# Autodesk Inventor assembly: BODY
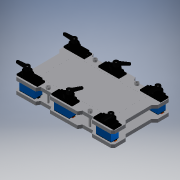
[picture p0: Inventor's stored thumbnail of the model, 180x180]
Saved by Autodesk Inventor 2017 (Build 210142000, 142)
## iProperties
Created: 2017-09-24
Part Number: BODY
Document SubType Name: Assembly
Designer: Alexander Miller
Author: Alexander Miller
## Documents named in this file (8)
- X:\Alex\Documents\Git\HeRo-Mini\Hardware\BODY.iam
- X:\Alex\Documents\Git\HeRo-Mini\Hardware\BODY_BOTTOM.ipt
- X:\Alex\Documents\Git\HeRo-Mini\Hardware\BODY_TOP.ipt
- X:\Alex\Documents\Git\HeRo-Mini\Hardware\SERVO.iam
- X:\Alex\Documents\Git\HeRo-Mini\Hardware\BODY_TOP_COVER.ipt
- X:\Alex\Documents\Git\HeRo-Mini\Hardware\MAGNET.ipt
- X:\Alex\Documents\Git\HeRo-Mini\Hardware\NUT_3MM.ipt
- X:\Alex\Documents\Git\HeRo-Mini\Hardware\M3_SCREW_25MM.ipt
## Components (35 placed, 7 different names)
1. BODY_BOTTOM:1 — Rigid:8, Rigid:9, Rigid:10, Rigid:11, Rigid:12, Rigid:13, Rigid:22, Rigid:23, Rigid:24, Rigid:25, Rigid:26, Rigid:27, Rigid:28, Rigid:29, Rigid:34, Rigid:35, Rigid:36, Rigid:37, Rigid:38, Rigid:39
2. BODY_TOP:1 — Rigid:7, Rigid:14, Rigid:15, Rigid:16, Rigid:17, Rigid:30, Rigid:31, Rigid:32, Rigid:33
3. SERVO:1 [sub-assembly] — Rigid:7, Rigid:13
4. SERVO:2 [sub-assembly] — Rigid:12
5. SERVO:3 [sub-assembly] — Rigid:11
6. SERVO:4 [sub-assembly] — Rigid:10
7. SERVO:5 [sub-assembly] — Rigid:9
8. SERVO:6 [sub-assembly] — Rigid:8
9. BODY_TOP_COVER:1 — Rigid:18, Rigid:19, Rigid:20, Rigid:21
10. MAGNET:1 — Rigid:15
11. MAGNET:2 — Rigid:16, Cylindrical:1
12. MAGNET:3 — Rigid:17
13. MAGNET:4 — Rigid:18, Cylindrical:1
14. MAGNET:5 — Rigid:14
15. MAGNET:6 — Rigid:20
16. MAGNET:7 — Rigid:21
17. MAGNET:8 — Rigid:19
18. NUT_3MM:1 — Rigid:22
19. NUT_3MM:2 — Rigid:24
20. NUT_3MM:3 — Rigid:26
21. NUT_3MM:4 — Rigid:23
22. NUT_3MM:5 — Rigid:27
23. NUT_3MM:6 — Rigid:25
24. NUT_3MM:7 — Rigid:29
25. NUT_3MM:8 — Rigid:28
26. M3_SCREW_25MM:1 — Rigid:30
27. M3_SCREW_25MM:2 — Rigid:31
28. M3_SCREW_25MM:3 — Rigid:32
29. M3_SCREW_25MM:4 — Rigid:33
30. NUT_3MM:9 — Rigid:35
31. NUT_3MM:10 — Rigid:34
32. NUT_3MM:11 — Rigid:36
33. NUT_3MM:12 — Rigid:37
34. NUT_3MM:13 — Rigid:39
35. NUT_3MM:14 — Rigid:38
## Relationships (34: WeldJoint 33, CylindricalJoint 1)
- Rigid:7 [WeldJoint]: BODY_TOP:1 ↔ SERVO:1
- Rigid:8 [WeldJoint]: BODY_BOTTOM:1 ↔ SERVO:6
- Rigid:9 [WeldJoint]: BODY_BOTTOM:1 ↔ SERVO:5
- Rigid:10 [WeldJoint]: BODY_BOTTOM:1 ↔ SERVO:4
- Rigid:11 [WeldJoint]: BODY_BOTTOM:1 ↔ SERVO:3
- Rigid:12 [WeldJoint]: BODY_BOTTOM:1 ↔ SERVO:2
- Rigid:13 [WeldJoint]: BODY_BOTTOM:1 ↔ SERVO:1
- Rigid:14 [WeldJoint]: BODY_TOP:1 ↔ MAGNET:5
- Rigid:15 [WeldJoint]: BODY_TOP:1 ↔ MAGNET:1
- Rigid:16 [WeldJoint]: BODY_TOP:1 ↔ MAGNET:2
- Rigid:17 [WeldJoint]: BODY_TOP:1 ↔ MAGNET:3
- Rigid:18 [WeldJoint]: BODY_TOP_COVER:1 ↔ MAGNET:4
- Rigid:19 [WeldJoint]: BODY_TOP_COVER:1 ↔ MAGNET:8
- Rigid:20 [WeldJoint]: BODY_TOP_COVER:1 ↔ MAGNET:6
- Rigid:21 [WeldJoint]: BODY_TOP_COVER:1 ↔ MAGNET:7
- Cylindrical:1: MAGNET:2 ↔ MAGNET:4
- Rigid:22 [WeldJoint]: BODY_BOTTOM:1 ↔ NUT_3MM:1
- Rigid:23 [WeldJoint]: BODY_BOTTOM:1 ↔ NUT_3MM:4
- Rigid:24 [WeldJoint]: BODY_BOTTOM:1 ↔ NUT_3MM:2
- Rigid:25 [WeldJoint]: BODY_BOTTOM:1 ↔ NUT_3MM:6
- Rigid:26 [WeldJoint]: BODY_BOTTOM:1 ↔ NUT_3MM:3
- Rigid:27 [WeldJoint]: BODY_BOTTOM:1 ↔ NUT_3MM:5
- Rigid:28 [WeldJoint]: BODY_BOTTOM:1 ↔ NUT_3MM:8
- Rigid:29 [WeldJoint]: BODY_BOTTOM:1 ↔ NUT_3MM:7
- Rigid:30 [WeldJoint]: BODY_TOP:1 ↔ M3_SCREW_25MM:1
- Rigid:31 [WeldJoint]: BODY_TOP:1 ↔ M3_SCREW_25MM:2
- Rigid:32 [WeldJoint]: BODY_TOP:1 ↔ M3_SCREW_25MM:3
- Rigid:33 [WeldJoint]: BODY_TOP:1 ↔ M3_SCREW_25MM:4
- Rigid:34 [WeldJoint]: BODY_BOTTOM:1 ↔ NUT_3MM:10
- Rigid:35 [WeldJoint]: BODY_BOTTOM:1 ↔ NUT_3MM:9
- Rigid:36 [WeldJoint]: BODY_BOTTOM:1 ↔ NUT_3MM:11
- Rigid:37 [WeldJoint]: BODY_BOTTOM:1 ↔ NUT_3MM:12
- Rigid:38 [WeldJoint]: BODY_BOTTOM:1 ↔ NUT_3MM:14
- Rigid:39 [WeldJoint]: BODY_BOTTOM:1 ↔ NUT_3MM:13
